# Autodesk Inventor assembly: Custom Cover Full Assembly_2
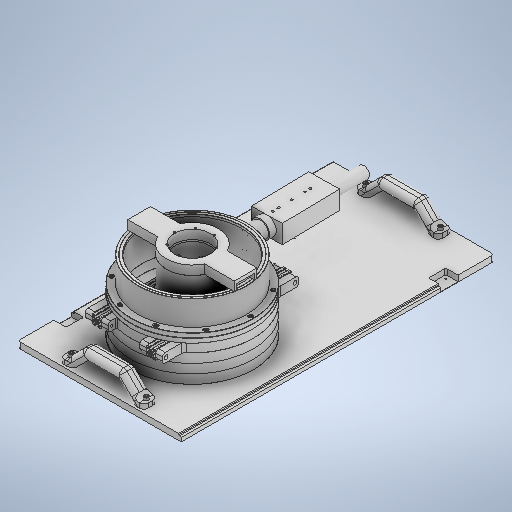
[picture p0: Inventor's stored thumbnail of the model, 512x512]
Saved by Autodesk Inventor 2025 (Build 290162000, 162)
## iProperties
Created: 2024-04-26
Part Number: Custom Cover Full Assembly_2
Document SubType Name: Assembly
Designer: Thienan Hoang
Author: Thienan Hoang
## Documents named in this file (15)
- C:\GitHub\In-situ-monitoring-of-powder-bed-fusion-additive-manufacturing\system_development\Orichalcum\v0.2\Hardware_design\custom-cover\Custom Cover Full Assembly_2.iam
- C:\GitHub\In-situ-monitoring-of-powder-bed-fusion-additive-manufacturing\system_development\Orichalcum\v0.2\Hardware_design\custom-cover\cover\Updated Cover.ipt
- C:\GitHub\In-situ-monitoring-of-powder-bed-fusion-additive-manufacturing\system_development\Orichalcum\v0.1\Hardware_design\galvo-scanner\GVS102.iam
- C:\GitHub\In-situ-monitoring-of-powder-bed-fusion-additive-manufacturing\system_development\Orichalcum\v0.2\Hardware_design\custom-cover\cylinder-parts\final-parts\Cylinder Slidey Bit.iam
- C:\GitHub\In-situ-monitoring-of-powder-bed-fusion-additive-manufacturing\system_development\Orichalcum\v0.2\Hardware_design\custom-cover\cylinder-parts\cylinder-segments\Head Thing.ipt
- C:\GitHub\In-situ-monitoring-of-powder-bed-fusion-additive-manufacturing\system_development\Orichalcum\v0.1\Hardware_design\custom-cover\cylinder-parts\final-parts\Cylinder Bottom.ipt
- C:\GitHub\In-situ-monitoring-of-powder-bed-fusion-additive-manufacturing\system_development\Orichalcum\v0.2\Hardware_design\custom-cover\cover\Handles.ipt
- C:\GitHub\In-situ-monitoring-of-powder-bed-fusion-additive-manufacturing\system_development\Orichalcum\v0.2\Hardware_design\custom-cover\8020-parts\ANSI B18.3.1M - M2x0.4 x 20(1).ipt
- C:\GitHub\In-situ-monitoring-of-powder-bed-fusion-additive-manufacturing\system_development\Orichalcum\v0.2\Hardware_design\custom-cover\8020-parts\ANSI B18.3.1M - M6x1 x 20(1).ipt
- C:\GitHub\In-situ-monitoring-of-powder-bed-fusion-additive-manufacturing\system_development\Orichalcum\v0.2\Hardware_design\custom-cover\8020-parts\ANSI B18.3.1M - M5x0.8 x 100(1).ipt
- C:\GitHub\In-situ-monitoring-of-powder-bed-fusion-additive-manufacturing\system_development\Orichalcum\v0.2\Hardware_design\custom-cover\cylinder-parts\Cylinder Spacer (x3).ipt
- C:\GitHub\In-situ-monitoring-of-powder-bed-fusion-additive-manufacturing\system_development\Orichalcum\v0.2\Hardware_design\custom-cover\cylinder-parts\Cylinder 80-20 Spacer_1.ipt
- C:\GitHub\In-situ-monitoring-of-powder-bed-fusion-additive-manufacturing\system_development\Orichalcum\v0.2\Hardware_design\custom-cover\cylinder-parts\Cylinder 80-20 Spacer_2.ipt
- C:\GitHub\In-situ-monitoring-of-powder-bed-fusion-additive-manufacturing\system_development\Orichalcum\v0.2\Hardware_design\custom-cover\8020-parts\20-2020-300.ipt
- C:\GitHub\In-situ-monitoring-of-powder-bed-fusion-additive-manufacturing\system_development\Orichalcum\v0.2\Hardware_design\laser-vibrometer\Updated Laser Scanner.ipt
## Components (38 placed, 14 different names)
1. Updated Cover:1 — Flush:5, Mate:48, Mate:98, Mate:106, Mate:107, Mate:108, Mate:109, Mate:128
2. GVS102:1 [sub-assembly]
3. Head Thing:1 — Mate:110, Mate:111, Insert:11, Insert:12, Insert:13, Insert:14, Insert:15, Insert:16, Insert:17
4. Cylinder Bottom:1 — Mate:98
5. Cylinder Slidey Bit:1 [sub-assembly] — Mate:110, Mate:111, Mate:112, Mate:113, Mate:114, Mate:115, Mate:116, Mate:117, Mate:118, Mate:119, Mate:120, Mate:121, Rigid:1
6. Handles:1 — Mate:108, Mate:109, Insert:18, Insert:19
7. Handles:2 — Mate:106, Mate:107, Insert:20, Insert:21
8. Cylinder Spacer (x3):1 — Rotational:1, Mate:128
9. Cylinder Spacer (x3):2 — Rotational:1, Rotational:2
10. Cylinder Spacer (x3):3 — Rotational:2, Mate:127
11. Cylinder 80-20 Spacer_1:1 — Flush:9, Flush:10, Mate:123, Mate:126, Flush:15, Flush:16
12. Cylinder 80-20 Spacer_2:1 — Mate:122, Flush:7, Flush:8
13. 20-2020-300:1 — Mate:122, Flush:7, Flush:8, Flush:9, Flush:10, Mate:123
14. Cylinder 80-20 Spacer_1:2
15. Cylinder 80-20 Spacer_2:2 — Mate:127
16. 20-2020-300:2 — Mate:126, Flush:15, Flush:16
17. Updated Laser Scanner:1 — Rigid:1
18. Forged Socket Head Cap Screw - Metric M2x0.4 x 20:1 — Insert:11
19. Forged Socket Head Cap Screw - Metric M2x0.4 x 20:2 — Insert:12
20. Forged Socket Head Cap Screw - Metric M2x0.4 x 20:3 — Insert:13
21. Forged Socket Head Cap Screw - Metric M2x0.4 x 20:4 — Insert:14
22. Forged Socket Head Cap Screw - Metric M2x0.4 x 20:5 — Insert:15
23. Forged Socket Head Cap Screw - Metric M2x0.4 x 20:6 — Insert:16
24. Forged Socket Head Cap Screw - Metric M2x0.4 x 20:7 — Insert:17
25. Forged Socket Head Cap Screw - Metric M6x1 x 20:1 — Insert:18
26. Forged Socket Head Cap Screw - Metric M6x1 x 20:2 — Insert:19
27. Forged Socket Head Cap Screw - Metric M6x1 x 20:3 — Insert:20
28. Forged Socket Head Cap Screw - Metric M6x1 x 20:4 — Insert:21
29. Forged Socket Head Cap Screw - Metric M5x0.8 x 100:1 — Mate:112
30. Forged Socket Head Cap Screw - Metric M5x0.8 x 100:3 — Mate:118
31. Forged Socket Head Cap Screw - Metric M5x0.8 x 100:4 — Mate:115
32. Forged Socket Head Cap Screw - Metric M5x0.8 x 100:5 — Mate:113
33. Forged Socket Head Cap Screw - Metric M5x0.8 x 100:6 — Mate:120
34. Forged Socket Head Cap Screw - Metric M5x0.8 x 100:7 — Mate:121
35. Forged Socket Head Cap Screw - Metric M5x0.8 x 100:8 — Mate:119
36. Forged Socket Head Cap Screw - Metric M5x0.8 x 100:9 — Mate:117
37. Forged Socket Head Cap Screw - Metric M5x0.8 x 100:10 — Mate:116
38. Forged Socket Head Cap Screw - Metric M5x0.8 x 100:11 — Mate:114
## Relationships (51: Mate 25, Flush 12, Insert 11, RevoluteJoint 2, WeldJoint 1)
- Flush:5 (180 mm): Updated Cover:1
- Mate:48: Updated Cover:1
- Flush:6 (38 mm)
- Mate:98: Updated Cover:1 ↔ Cylinder Bottom:1
- Mate:106: Updated Cover:1 ↔ Handles:2
- Mate:107: Updated Cover:1 ↔ Handles:2
- Mate:108: Updated Cover:1 ↔ Handles:1
- Mate:109: Updated Cover:1 ↔ Handles:1
- Mate:110: Head Thing:1 ↔ Cylinder Slidey Bit:1
- Mate:111: Head Thing:1 ↔ Cylinder Slidey Bit:1
- Insert:11: Head Thing:1 ↔ Forged Socket Head Cap Screw - Metric M2x0.4 x 20:1
- Insert:12: Head Thing:1 ↔ Forged Socket Head Cap Screw - Metric M2x0.4 x 20:2
- Insert:13: Head Thing:1 ↔ Forged Socket Head Cap Screw - Metric M2x0.4 x 20:3
- Insert:14: Head Thing:1 ↔ Forged Socket Head Cap Screw - Metric M2x0.4 x 20:4
- Insert:15: Head Thing:1 ↔ Forged Socket Head Cap Screw - Metric M2x0.4 x 20:5
- Insert:16: Head Thing:1 ↔ Forged Socket Head Cap Screw - Metric M2x0.4 x 20:6
- Insert:17: Head Thing:1 ↔ Forged Socket Head Cap Screw - Metric M2x0.4 x 20:7
- Insert:18: Handles:1 ↔ Forged Socket Head Cap Screw - Metric M6x1 x 20:1
- Insert:19: Handles:1 ↔ Forged Socket Head Cap Screw - Metric M6x1 x 20:2
- Insert:20: Handles:2 ↔ Forged Socket Head Cap Screw - Metric M6x1 x 20:3
- Insert:21: Handles:2 ↔ Forged Socket Head Cap Screw - Metric M6x1 x 20:4
- Mate:112: Cylinder Slidey Bit:1 ↔ Forged Socket Head Cap Screw - Metric M5x0.8 x 100:1
- Mate:113: Cylinder Slidey Bit:1 ↔ Forged Socket Head Cap Screw - Metric M5x0.8 x 100:5
- Mate:114: Cylinder Slidey Bit:1 ↔ Forged Socket Head Cap Screw - Metric M5x0.8 x 100:11
- Mate:115: Cylinder Slidey Bit:1 ↔ Forged Socket Head Cap Screw - Metric M5x0.8 x 100:4
- Mate:116: Cylinder Slidey Bit:1 ↔ Forged Socket Head Cap Screw - Metric M5x0.8 x 100:10
- Mate:117: Cylinder Slidey Bit:1 ↔ Forged Socket Head Cap Screw - Metric M5x0.8 x 100:9
- Mate:118: Cylinder Slidey Bit:1 ↔ Forged Socket Head Cap Screw - Metric M5x0.8 x 100:3
- Mate:119: Cylinder Slidey Bit:1 ↔ Forged Socket Head Cap Screw - Metric M5x0.8 x 100:8
- Mate:120: Cylinder Slidey Bit:1 ↔ Forged Socket Head Cap Screw - Metric M5x0.8 x 100:6
- Mate:121: Cylinder Slidey Bit:1 ↔ Forged Socket Head Cap Screw - Metric M5x0.8 x 100:7
- Rotational:1 [RevoluteJoint]: Cylinder Spacer (x3):1 ↔ Cylinder Spacer (x3):2
- Rotational:2 [RevoluteJoint]: Cylinder Spacer (x3):2 ↔ Cylinder Spacer (x3):3
- Mate:122: Cylinder 80-20 Spacer_2:1 ↔ 20-2020-300:1
- Flush:7: Cylinder 80-20 Spacer_2:1 ↔ 20-2020-300:1
- Flush:8: Cylinder 80-20 Spacer_2:1 ↔ 20-2020-300:1
- Flush:9: Cylinder 80-20 Spacer_1:1 ↔ 20-2020-300:1
- Flush:10: Cylinder 80-20 Spacer_1:1 ↔ 20-2020-300:1
- Mate:123: Cylinder 80-20 Spacer_1:1 ↔ 20-2020-300:1
- [Mate]: Cylinder 80-20 Spacer_2:2 ↔ 20-2020-300:2
- [Flush]: Cylinder 80-20 Spacer_2:2 ↔ 20-2020-300:2
- [Flush]: Cylinder 80-20 Spacer_2:2 ↔ 20-2020-300:2
- [Flush]: Cylinder 80-20 Spacer_1:2 ↔ 20-2020-300:2
- [Flush]: Cylinder 80-20 Spacer_1:2 ↔ 20-2020-300:2
- [Mate]: Cylinder 80-20 Spacer_1:2 ↔ 20-2020-300:2
- Mate:126: Cylinder 80-20 Spacer_1:1 ↔ 20-2020-300:2
- Flush:15: Cylinder 80-20 Spacer_1:1 ↔ 20-2020-300:2
- Flush:16: Cylinder 80-20 Spacer_1:1 ↔ 20-2020-300:2
- Mate:127: Cylinder Spacer (x3):3 ↔ Cylinder 80-20 Spacer_2:2
- Mate:128: Updated Cover:1 ↔ Cylinder Spacer (x3):1
- Rigid:1 [WeldJoint]: Cylinder Slidey Bit:1 ↔ Updated Laser Scanner:1
## Named parameters: d405_d399 = 0 mm, d406_d400 = 0 mm, d407_d401 = 0 mm, d408_d402 = 0 mm, d409_d403 = 0 mm, d410_d404 = 0 mm
